# Autodesk Inventor assembly: 615468_double_spool_Assembly
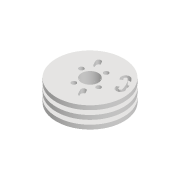
[picture p0: Inventor's stored thumbnail of the model, 180x180]
Saved by Autodesk Inventor 2020 (Build 240168000, 168)
## iProperties
Created: 2019-11-26
Part Number: 615468_double_spool_Assembly
Document SubType Name: Assembly
Designer: ball
Author: ball
## Documents named in this file (3)
- C:\FTC\FTC8863CAD\Actobotics\565 parts\615468_double_spool_Assembly.iam
- C:\FTC\FTC8863CAD\Actobotics\615 parts\615468 outer plate.ipt
- C:\FTC\FTC8863CAD\Actobotics\615 parts\615468 inner plate.ipt
## Components (5 placed, 2 different names)
1. 615468 outer plate:1 — Mate:1, Mate:2, Mate:3
2. 615468 inner plate:1 — Mate:1, Mate:2, Mate:3, Mate:4, Mate:5, Mate:6, Mate:8
3. 615468 outer plate:2 — Mate:4, Mate:5, Mate:6, Mate:7, Mate:9
4. 615468 outer plate:3 — Mate:10, Mate:11, Mate:12
5. 615468 inner plate:2 — Mate:7, Mate:8, Mate:9, Mate:10, Mate:11, Mate:12
## Relationships (12: Mate 12)
- Mate:1: 615468 outer plate:1 ↔ 615468 inner plate:1
- Mate:2: 615468 outer plate:1 ↔ 615468 inner plate:1
- Mate:3: 615468 outer plate:1 ↔ 615468 inner plate:1
- Mate:4: 615468 inner plate:1 ↔ 615468 outer plate:2
- Mate:5: 615468 inner plate:1 ↔ 615468 outer plate:2
- Mate:6: 615468 inner plate:1 ↔ 615468 outer plate:2
- Mate:7: 615468 outer plate:2 ↔ 615468 inner plate:2
- Mate:8: 615468 inner plate:1 ↔ 615468 inner plate:2
- Mate:9: 615468 outer plate:2 ↔ 615468 inner plate:2
- Mate:10: 615468 outer plate:3 ↔ 615468 inner plate:2
- Mate:11: 615468 outer plate:3 ↔ 615468 inner plate:2
- Mate:12: 615468 outer plate:3 ↔ 615468 inner plate:2
